# Autodesk Inventor assembly: Holder_m_base
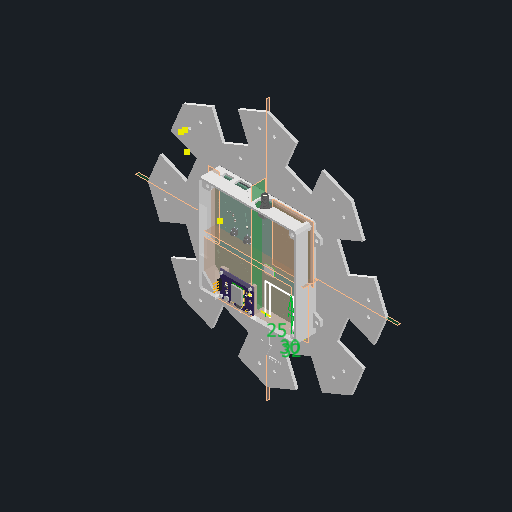
[picture p0: Inventor's stored thumbnail of the model, 512x512]
Saved by Autodesk Inventor 2026.2 (Build 302298000, 298)
## iProperties
Created: 2026-04-25
Part Number: Holder_m_base
Document SubType Name: Assembly
Designer: Malthe Sennels
Author: Malthe Sennels
## Documents named in this file (8)
- C:\Users\Malthe Sennels\OneDrive - Aalborg Universitet\ESD 610 - General\Inventor\Drone_holder_v2\Holder_m_base.iam
- C:\Users\Malthe Sennels\OneDrive - Aalborg Universitet\ESD 610 - General\Inventor\Drone_holder_v2\Drone_modem.ipt
- C:\Users\Malthe Sennels\OneDrive - Aalborg Universitet\ESD 610 - General\Inventor\Drone_holder_v2\Buttom_part.ipt
- C:\Users\Malthe Sennels\OneDrive - Aalborg Universitet\ESD 610 - General\Inventor\Drone_holder_v2\GPS.ipt
- C:\Users\Malthe Sennels\OneDrive - Aalborg Universitet\ESD 610 - General\Inventor\Drone_holder_v2\Buttom_acrylic.ipt
- C:\Users\Malthe Sennels\OneDrive - Aalborg Universitet\ESD 610 - General\Inventor\Drone_holder_v2\Lid_1.ipt
- C:\Users\Malthe Sennels\OneDrive - Aalborg Universitet\ESD 610 - General\Inventor\Drone_holder_v2\Bund.ipt
- C:\Users\Malthe Sennels\OneDrive - Aalborg Universitet\ESD 610 - General\Inventor\Drone_holder_v2\Lid_clear.ipt
## Components (7 placed, 7 different names)
1. Drone_modem:1 — Mate:1, Flush:1, Mate:2, Flush:2, Flush:4, Flush:6, Mate:5
2. Buttom_part:1 — Flush:2, Flush:3, Mate:3, Mate:4, Angle:1, Flush:5, Flush:8, Flush:9, Flush:10, Flush:11, Flush:12
3. GPS:1 — Mate:3, Mate:4, Angle:1
4. Buttom_acrylic:1 — Flush:3, Flush:7
5. Lid_1:1 — Flush:4, Flush:5, Flush:8, Flush:9, Flush:10, Flush:11, Flush:12, Flush:13
6. Bund:1 — Flush:6, Mate:5, Flush:7
7. Lid_clear:1 — Flush:13
## Relationships (19: Flush 13, Mate 5, Angle 1)
- Mate:1: Drone_modem:1
- Flush:1: Drone_modem:1
- Mate:2: Drone_modem:1
- Flush:2: Drone_modem:1 ↔ Buttom_part:1
- Flush:3: Buttom_part:1 ↔ Buttom_acrylic:1
- Mate:3: Buttom_part:1 ↔ GPS:1
- Mate:4: Buttom_part:1 ↔ GPS:1
- Angle:1 (0 deg): Buttom_part:1 ↔ GPS:1
- Flush:4: Drone_modem:1 ↔ Lid_1:1
- Flush:5: Buttom_part:1 ↔ Lid_1:1
- Flush:6: Drone_modem:1 ↔ Bund:1
- Mate:5: Drone_modem:1 ↔ Bund:1
- Flush:7: Buttom_acrylic:1 ↔ Bund:1
- Flush:8: Buttom_part:1 ↔ Lid_1:1
- Flush:9: Buttom_part:1 ↔ Lid_1:1
- Flush:10: Buttom_part:1 ↔ Lid_1:1
- Flush:11: Buttom_part:1 ↔ Lid_1:1
- Flush:12: Buttom_part:1 ↔ Lid_1:1
- Flush:13: Lid_1:1 ↔ Lid_clear:1
